# Autodesk Inventor assembly: Slider_crank_mechanism
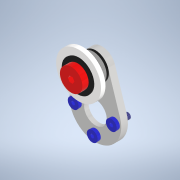
[picture p0: Inventor's stored thumbnail of the model, 180x180]
Saved by Autodesk Inventor 2020.4 (Build 244396000, 396)
## iProperties
Created: 2021-09-06
Part Number: Slider_crank_mechanism
Document SubType Name: Assembly
Designer: Masato Kubotera
Mass: 2.53036 g
Surface Area: 18.5815 cm^2
Volume: 1.13409 cm^3
Density: 2.23118 g/cm^3
Author: Masato Kubotera
## Documents named in this file (9)
- C:\Users\Masato\Documents\Inventor\CIT Brains_Inventor\OpenPlatform_ver3_0 - ve4_1 branch\LowerBody\Slider_crank\Slider_crank_mechanism.iam
- C:\Users\Masato\Documents\Inventor\CIT Brains_Inventor\OpenPlatform_ver3_0 - ve4_1 branch\LowerBody\Slider_crank\Slider_crank_horn.ipt
- C:\Users\Masato\Documents\Inventor\CIT Brains_Inventor\OpenPlatform_ver3_0 - ve4_1 branch\Ready_Made\LED-0606.ipt
- C:\Users\Masato\Documents\Inventor\CIT Brains_Inventor\OpenPlatform_ver3_0 - ve4_1 branch\Ready_Made\Screw\M2_6-6.ipt
- C:\Users\Masato\Documents\Inventor\CIT Brains_Inventor\OpenPlatform_ver3_0 - ve4_1 branch\Ready_Made\TT-1020-20.ipt
- C:\Users\Masato\Documents\Inventor\CIT Brains_Inventor\OpenPlatform_ver3_0 - ve4_1 branch\Ready_Made\UUW-0412-10BH.ipt
- C:\Users\Masato\Documents\Inventor\CIT Brains_Inventor\OpenPlatform_ver3_0 - ve4_1 branch\Ready_Made\InsertNut\S4-05-3W.ipt
- C:\Users\Masato\Documents\Inventor\CIT Brains_Inventor\OpenPlatform_ver3_0 - ve4_1 branch\Ready_Made\UUW-0614-05BH.ipt
- C:\Users\Masato\Documents\Inventor\CIT Brains_Inventor\OpenPlatform_ver3_0 - ve4_1 branch\Ready_Made\DBS4-7-4.ipt
## Components (11 placed, 8 different names)
1. Slider_crank_horn:1 — 挿入:1, 角度:1, 挿入:2, 挿入:3, 挿入:4, 挿入:5, 挿入:6, 角度:2, フラッシュ:1, フラッシュ:2, フラッシュ:3
2. M2_6-6:1 — 挿入:3
3. M2_6-6:2 — 挿入:5
4. M2_6-6:3 — 挿入:4
5. M2_6-6:4 — 挿入:6
6. UUW-0412-10BH:1 — 挿入:7, 挿入:2, 挿入:8
7. LED-0606:1 — 挿入:7, 角度:2
8. TT-1020-20:1 — 挿入:10
9. S4-05-3W:1 — 角度:1, 挿入:1
10. UUW-0614-05BH:1 — 挿入:9, 挿入:10
11. DBS4-7-4:1 — 挿入:8, 挿入:9
## Relationships (15: Insert 10, Flush 3, Angle 2)
- 挿入:1 [Insert]: Slider_crank_horn:1 ↔ S4-05-3W:1
- 角度:1 [Angle] (0 deg): Slider_crank_horn:1 ↔ S4-05-3W:1
- 挿入:2 [Insert]: Slider_crank_horn:1 ↔ UUW-0412-10BH:1
- 挿入:3 [Insert]: Slider_crank_horn:1 ↔ M2_6-6:1
- 挿入:4 [Insert]: Slider_crank_horn:1 ↔ M2_6-6:3
- 挿入:5 [Insert]: Slider_crank_horn:1 ↔ M2_6-6:2
- 挿入:6 [Insert]: Slider_crank_horn:1 ↔ M2_6-6:4
- 挿入:7 [Insert]: UUW-0412-10BH:1 ↔ LED-0606:1
- 挿入:8 [Insert]: UUW-0412-10BH:1 ↔ DBS4-7-4:1
- 挿入:9 [Insert]: UUW-0614-05BH:1 ↔ DBS4-7-4:1
- 挿入:10 [Insert]: TT-1020-20:1 ↔ UUW-0614-05BH:1
- 角度:2 [Angle] (0 deg): Slider_crank_horn:1 ↔ LED-0606:1
- フラッシュ:1 [Flush]: Slider_crank_horn:1
- フラッシュ:2 [Flush]: Slider_crank_horn:1
- フラッシュ:3 [Flush]: Slider_crank_horn:1
